# Autodesk Inventor assembly: Planetery gearbox
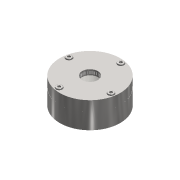
[picture p0: Inventor's stored thumbnail of the model, 180x180]
Saved by Autodesk Inventor 2020.3 (Build 243373010, 373A)
## iProperties
Created: 2021-05-04
Part Number: Planetery gearbox
Document SubType Name: Assembly
Designer: marti
Author: marti
## Documents named in this file (12)
- C:\Users\marti\Documents\Inventor\RobotManipulateArm\17.4.2021 - Complete new IDEA\Planetery gearbox.iam
- C:\Users\marti\Documents\Inventor\RobotManipulateArm\17.4.2021 - Complete new IDEA\Planetery gearbox\Design Accelerator\Spur Gears5.iam
- C:\Users\marti\Documents\Inventor\RobotManipulateArm\17.4.2021 - Complete new IDEA\Planetery gearbox\Design Accelerator\Spur Gears9.iam
- C:\Users\marti\Documents\Inventor\RobotManipulateArm\17.4.2021 - Complete new IDEA\Planetery gearbox\Design Accelerator\Spur Gears10.iam
- C:\Users\marti\Documents\Inventor\RobotManipulateArm\17.4.2021 - Complete new IDEA\Planetery gearbox port.ipt
- C:\Users\marti\Documents\Inventor\RobotManipulateArm\17.4.2021 - Complete new IDEA\Planetery gearbox\Design Accelerator\Bearing1.iam
- C:\Users\marti\Documents\Inventor\RobotManipulateArm\17.4.2021 - Complete new IDEA\Cover of port.ipt
- C:\Users\marti\Documents\Inventor\Content Center Files\R2020\en-US\ISO 4762(1)\DIN EN ISO 4762 - M2 x 10.ipt
- C:\Users\marti\Documents\Inventor\RobotManipulateArm\17.4.2021 - Complete new IDEA\Housing of planetary gearbox.ipt
- C:\Users\marti\Documents\Inventor\RobotManipulateArm\17.4.2021 - Complete new IDEA\Housing of planetary gearbox part 2.ipt
- C:\Users\marti\Documents\Inventor\RobotManipulateArm\17.4.2021 - Complete new IDEA\Inner disc of housing of gearbox.ipt
- C:\Users\marti\Documents\Inventor\Content Center Files\R2020\en-US\ISO 4762(1)\DIN EN ISO 4762 - M3 x 16.ipt
## Components (25 placed, 9 different names)
1. Spur Gears:1 [sub-assembly] — Flush:6, Angle:18, Mate:16, Rotation:6, Mate:18, Flush:10, Flush:14
2. Spur Gears:2 [sub-assembly] — Mate:10, Mate:11, Flush:5, Flush:6, Mate:13, Flush:7, Flush:8, Rotation:3, Angle:19, Angle:20, Angle:18, Rotation:6, Rotation:7, Rotation:8, Rotation:9, Mate:38, Mate:40, Mate:42
3. Spur Gears:3 [sub-assembly] — Mate:11, Flush:5, Rotation:3, Mate:41, Mate:56
4. Planetery gearbox port:1 — Mate:7, Flush:3, Mate:10, Mate:13, Mate:14, Mate:15, Mate:16, Rotation:9, Mate:20, Mate:21, Mate:22, Mate:23, Mate:25, Mate:27
5. Spur Gears:4 [sub-assembly] — Flush:7, Angle:19, Mate:14, Rotation:7, Mate:19, Flush:11, Flush:12
6. Spur Gears:5 [sub-assembly] — Flush:8, Mate:15, Mate:17, Flush:9, Angle:20, Rotation:8, Flush:13
7. Bearing:1 [sub-assembly] — Mate:17, Flush:9
8. Bearing:2 [sub-assembly] — Mate:18, Flush:10
9. Bearing:3 [sub-assembly] — Mate:19, Flush:11
10. Bearing:4 [sub-assembly] — Mate:22, Flush:14, Mate:26
11. Bearing:5 [sub-assembly] — Mate:20, Flush:12, Mate:28
12. Bearing:6 [sub-assembly] — Mate:21, Flush:13, Mate:24
13. Cover of port:1 — Mate:23, Mate:28, Mate:31, Mate:32, Mate:37
14. Cover of port:2 — Mate:24, Mate:25, Mate:29, Mate:30
15. Cover of port:3 — Mate:26, Mate:27, Mate:33, Mate:34
16. DIN EN ISO 4762 M2 x 10:1 — Mate:31, Mate:32
17. DIN EN ISO 4762 M2 x 10:2 — Mate:29, Mate:30
18. DIN EN ISO 4762 M2 x 10:3 — Mate:33, Mate:34
19. Housing of planetary gearbox:1 — Mate:42, Mate:43, Mate:44, Mate:46, Mate:47, Mate:48, Mate:49, Mate:50, Mate:51, Mate:52, Mate:53, Mate:54, Mate:55
20. Housing of planetary gearbox part 2:1 — Mate:40, Mate:41, Mate:43, Mate:44, Mate:46
21. Inner disc of housing of gearbox:1 — Mate:37, Mate:38, Mate:56
22. DIN EN ISO 4762 M3 x 16:2 — Mate:52, Mate:53
23. DIN EN ISO 4762 M3 x 16:3 — Mate:50, Mate:51
24. DIN EN ISO 4762 M3 x 16:5 — Mate:48, Mate:49
25. DIN EN ISO 4762 M3 x 16:6 — Mate:54, Mate:55
## Relationships (62: Mate 43, Flush 11, RelateRotation 5, Angle 3)
- Mate:7: Planetery gearbox port:1
- Flush:3: Planetery gearbox port:1
- Mate:10: Spur Gears:2 ↔ Planetery gearbox port:1
- Mate:11: Spur Gears:2 ↔ Spur Gears:3
- Flush:5: Spur Gears:2 ↔ Spur Gears:3
- Flush:6: Spur Gears:1 ↔ Spur Gears:2
- Mate:13: Spur Gears:2 ↔ Planetery gearbox port:1
- Flush:7: Spur Gears:2 ↔ Spur Gears:4
- Flush:8: Spur Gears:2 ↔ Spur Gears:5
- Angle:18 (0 deg): Spur Gears:1 ↔ Spur Gears:2
- Rotation:3 [RelateRotation] (2 ul): Spur Gears:2 ↔ Spur Gears:3
- Angle:19 (0 deg): Spur Gears:2 ↔ Spur Gears:4
- Mate:14: Planetery gearbox port:1 ↔ Spur Gears:4
- Mate:15: Planetery gearbox port:1 ↔ Spur Gears:5
- Mate:16: Spur Gears:1 ↔ Planetery gearbox port:1
- Rotation:6 [RelateRotation] (0.2 ul): Spur Gears:1 ↔ Spur Gears:2
- Rotation:7 [RelateRotation] (0.2 ul): Spur Gears:2 ↔ Spur Gears:4
- Rotation:9 [RelateRotation] (1 ul): Spur Gears:2 ↔ Planetery gearbox port:1
- Mate:17: Spur Gears:5 ↔ Bearing:1
- Flush:9: Spur Gears:5 ↔ Bearing:1
- Angle:20 (0 deg): Spur Gears:2 ↔ Spur Gears:5
- Rotation:8 [RelateRotation] (0.2 ul): Spur Gears:2 ↔ Spur Gears:5
- Mate:18: Spur Gears:1 ↔ Bearing:2
- Flush:10: Spur Gears:1 ↔ Bearing:2
- Mate:19: Spur Gears:4 ↔ Bearing:3
- Flush:11: Spur Gears:4 ↔ Bearing:3
- Mate:20: Planetery gearbox port:1 ↔ Bearing:5
- Flush:12: Spur Gears:4 ↔ Bearing:5
- Mate:21: Planetery gearbox port:1 ↔ Bearing:6
- Flush:13: Spur Gears:5 ↔ Bearing:6
- Mate:22: Planetery gearbox port:1 ↔ Bearing:4
- Flush:14: Spur Gears:1 ↔ Bearing:4
- Mate:23: Planetery gearbox port:1 ↔ Cover of port:1
- Mate:24: Bearing:6 ↔ Cover of port:2
- Mate:25: Planetery gearbox port:1 ↔ Cover of port:2
- Mate:26: Bearing:4 ↔ Cover of port:3
- Mate:27: Planetery gearbox port:1 ↔ Cover of port:3
- Mate:28: Bearing:5 ↔ Cover of port:1
- Mate:29: Cover of port:2 ↔ DIN EN ISO 4762 M2 x 10:2
- Mate:30: Cover of port:2 ↔ DIN EN ISO 4762 M2 x 10:2
- Mate:31: Cover of port:1 ↔ DIN EN ISO 4762 M2 x 10:1
- Mate:32: Cover of port:1 ↔ DIN EN ISO 4762 M2 x 10:1
- Mate:33: Cover of port:3 ↔ DIN EN ISO 4762 M2 x 10:3
- Mate:34: Cover of port:3 ↔ DIN EN ISO 4762 M2 x 10:3
- Mate:37: Cover of port:1 ↔ Inner disc of housing of gearbox:1
- Mate:38: Spur Gears:2 ↔ Inner disc of housing of gearbox:1
- Mate:40: Spur Gears:2 ↔ Housing of planetary gearbox part 2:1
- Mate:41: Spur Gears:3 ↔ Housing of planetary gearbox part 2:1
- Mate:42: Spur Gears:2 ↔ Housing of planetary gearbox:1
- Mate:43: Housing of planetary gearbox:1 ↔ Housing of planetary gearbox part 2:1
- Mate:44: Housing of planetary gearbox:1 ↔ Housing of planetary gearbox part 2:1
- Mate:46: Housing of planetary gearbox:1 ↔ Housing of planetary gearbox part 2:1
- Mate:47: Housing of planetary gearbox:1
- Mate:48: Housing of planetary gearbox:1 ↔ DIN EN ISO 4762 M3 x 16:5
- Mate:49: Housing of planetary gearbox:1 ↔ DIN EN ISO 4762 M3 x 16:5
- Mate:50: Housing of planetary gearbox:1 ↔ DIN EN ISO 4762 M3 x 16:3
- Mate:51: Housing of planetary gearbox:1 ↔ DIN EN ISO 4762 M3 x 16:3
- Mate:52: Housing of planetary gearbox:1 ↔ DIN EN ISO 4762 M3 x 16:2
- Mate:53: Housing of planetary gearbox:1 ↔ DIN EN ISO 4762 M3 x 16:2
- Mate:54: Housing of planetary gearbox:1 ↔ DIN EN ISO 4762 M3 x 16:6
- Mate:55: Housing of planetary gearbox:1 ↔ DIN EN ISO 4762 M3 x 16:6
- Mate:56: Spur Gears:3 ↔ Inner disc of housing of gearbox:1
